# Autodesk Inventor assembly: StrainWaveGearbox
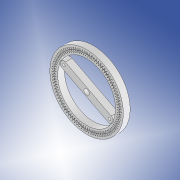
[picture p0: Inventor's stored thumbnail of the model, 180x180]
Saved by Autodesk Inventor 2017 (Build 210142000, 142)
## iProperties
Created: 2017-07-11
Part Number: StrainWaveGearbox
Document SubType Name: Assembly
Designer: zallen
Author: zallen
## Documents named in this file (4)
- C:\Users\zallen\Documents\GitHub\cr-laundry-robot\lib\Strain Wave Gearbox\StrainWaveGearbox.iam
- C:\Users\zallen\Documents\GitHub\cr-laundry-robot\lib\Strain Wave Gearbox\Flexspline.ipt
- C:\Users\zallen\Documents\GitHub\cr-laundry-robot\lib\Strain Wave Gearbox\Basespline.ipt
- C:\Users\zallen\Documents\GitHub\cr-laundry-robot\lib\Strain Wave Gearbox\WaveGenerator.ipt
## Components (3 placed, 3 different names)
1. Flexspline:1 — Mate:1, Flush:1
2. Basespline:1 — Mate:1, Flush:1, Flush:2, Mate:2, Mate:3, Mate:4, Flush:3, Rotation:1
3. WaveGenerator:1 — Mate:4, Flush:3, Rotation:1
## Relationships (8: Mate 4, Flush 3, RelateRotation 1)
- Mate:1: Flexspline:1 ↔ Basespline:1
- Flush:1: Flexspline:1 ↔ Basespline:1
- Flush:2: Basespline:1
- Mate:2: Basespline:1
- Mate:3: Basespline:1
- Mate:4: Basespline:1 ↔ WaveGenerator:1
- Flush:3: Basespline:1 ↔ WaveGenerator:1
- Rotation:1 [RelateRotation] (0.0217 ul): Basespline:1 ↔ WaveGenerator:1
